# Autodesk Inventor assembly: BINDER CLIP
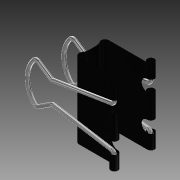
[picture p0: Inventor's stored thumbnail of the model, 180x180]
Saved by Autodesk Inventor 2013 (Build 170138000, 138)
## iProperties
Created: 2014-06-22
Part Number: BINDER CLIP
Document SubType Name: Assembly
Designer: employee
Author: employee
## Documents named in this file (3)
- C:\Users\employee\Desktop\CoreXZ 2\BINDER CLIP.iam
- C:\Users\employee\Desktop\CoreXZ 2\BINDER CLIP BODY.ipt
- C:\Users\employee\Desktop\CoreXZ 2\BINDER CLIP ARM.ipt
## Components (3 placed, 2 different names)
1. BINDER CLIP BODY:1 — Insert:1, Insert:2, Angle:1, Angle:2
2. BINDER CLIP ARM:1 — Insert:1, Angle:1
3. BINDER CLIP ARM:2 — Insert:2, Angle:2
## Relationships (4: Insert 2, Angle 2)
- Insert:1: BINDER CLIP BODY:1 ↔ BINDER CLIP ARM:1
- Insert:2: BINDER CLIP BODY:1 ↔ BINDER CLIP ARM:2
- Angle:1 (0 deg): BINDER CLIP BODY:1 ↔ BINDER CLIP ARM:1
- Angle:2 (0 deg): BINDER CLIP BODY:1 ↔ BINDER CLIP ARM:2
